# Autodesk Inventor assembly: First Base Extension (Draft 2)
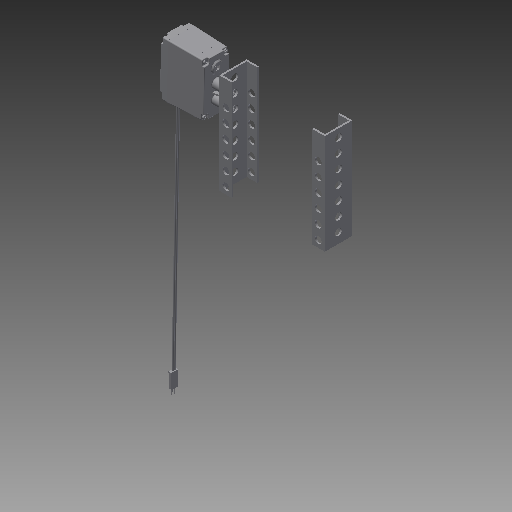
[picture p0: Inventor's stored thumbnail of the model, 512x512]
Saved by Autodesk Inventor 2018 (Build 220112000, 112)
## iProperties
Created: 2017-06-28
Part Number: First Base Extension (Draft 2)
Document SubType Name: Assembly
Designer: James
Author: James
## Documents named in this file (3)
- C:\Users\James\Desktop\EE REU\Hardware\Vex Arm\Vex Arm Draft 2\First Base Extension (Draft 2).iam
- C:\Users\James\Desktop\EE REU\Hardware\Vex Arm\Vex Parts\Base C Channel.ipt
- C:\Users\James\Desktop\EE REU\Hardware\Vex Arm\Vex Parts\393motor.ipt
## Components (3 placed, 2 different names)
1. Base C Channel:1 — Mate:1, Flush:1, Flush:2, Insert:1
2. Base C Channel:2 — Mate:1, Flush:1, Flush:2
3. 393motor:1 — Insert:1
## Relationships (4: Flush 2, Mate 1, Insert 1)
- Mate:1 (94.996 mm): Base C Channel:1 ↔ Base C Channel:2
- Flush:1: Base C Channel:1 ↔ Base C Channel:2
- Flush:2: Base C Channel:1 ↔ Base C Channel:2
- Insert:1: Base C Channel:1 ↔ 393motor:1
